# Autodesk Inventor assembly: Сборка
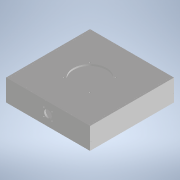
[picture p0: Inventor's stored thumbnail of the model, 180x180]
Saved by Autodesk Inventor 2021 (Build 250183000, 183)
## iProperties
Created: 2021-04-10
Part Number: Сборка
Document SubType Name: Assembly
Designer: user
Author: user
## Documents named in this file (6)
- C:\Users\user.DESKTOP-BLHF870\Documents\Турель\Сборка.iam
- C:\Users\user.DESKTOP-BLHF870\Documents\Турель\Верх.ipt
- C:\Users\user.DESKTOP-BLHF870\Documents\Турель\Стекнка t1.ipt
- C:\Users\user.DESKTOP-BLHF870\Documents\Турель\Стекнка t2.ipt
- C:\Users\user.DESKTOP-BLHF870\Documents\Турель\Стекнка t3.ipt
- C:\Users\user.DESKTOP-BLHF870\Documents\Турель\Низ.ipt
## Components (6 placed, 5 different names)
1. Верх:1 — Жесткий:1, Жесткий:2, Жесткий:3, Жесткий:4
2. Стекнка t1:1 — Жесткий:2
3. Стекнка t1:2 — Жесткий:1
4. Стекнка t2:1 — Жесткий:3, Жесткий:5
5. Стекнка t3:1 — Жесткий:4
6. Низ:1 — Жесткий:5
## Relationships (5: WeldJoint 5)
- Жесткий:1 [WeldJoint]: Верх:1 ↔ Стекнка t1:2
- Жесткий:2 [WeldJoint]: Верх:1 ↔ Стекнка t1:1
- Жесткий:3 [WeldJoint]: Верх:1 ↔ Стекнка t2:1
- Жесткий:4 [WeldJoint]: Верх:1 ↔ Стекнка t3:1
- Жесткий:5 [WeldJoint]: Стекнка t2:1 ↔ Низ:1
